# Autodesk Inventor assembly: PCB enclosure_v2
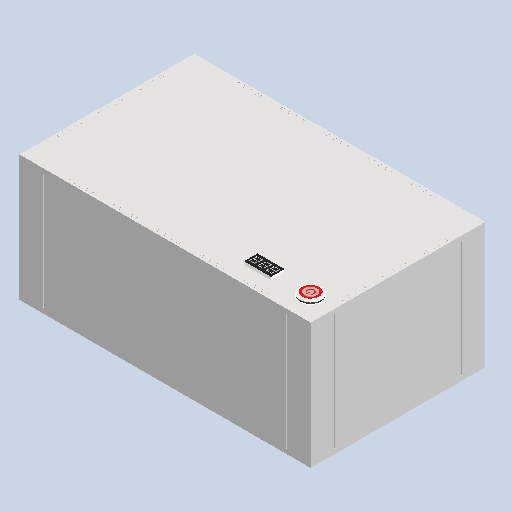
[picture p0: Inventor's stored thumbnail of the model, 512x512]
Saved by Autodesk Inventor 2026 (Build 300175050, 175E)
## iProperties
Created: 2025-10-28
Part Number: PCB enclosure_v2
Document SubType Name: Assembly
Designer: Kartik
Mass: 882.1 g
Surface Area: 6140.05 cm^2
Volume: 881.115 cm^3
Density: 1.00112 g/cm^3
Author: Kartik
## Documents named in this file (18)
- D:\Kartik\Projects\AMR\CAD\2 Sub-assembly\PCB enclosure_v2.iam
- D:\Kartik\Projects\AMR\CAD\4 Boughtouts\MDD20A CAD\MDD20A\MDD20A\MDD20A.ipt
- D:\Kartik\Projects\AMR\CAD\4 Boughtouts\NUCLEO-F401RE--3DModel-STEP-56544\NUCLEO-F401RE--3DModel-STEP-56544\NUCLEO-F401RE--3DModel-STEP-56544.ipt
- D:\Kartik\Projects\AMR\CAD\4 Boughtouts\nvidia-jetson-nano-4gb\Jetson nano 4GB\Jetson nano 4GB\Jetson nano 4GB.ipt
- D:\Kartik\Projects\AMR\CAD\4 Boughtouts\arduino-uno-screw-shield-1\Arduino Uno Screw Shield\Arduino Uno Screw Shield\Arduino Uno Screw Shield.ipt
- D:\Kartik\Projects\AMR\CAD\4 Boughtouts\xh-m401-buck-converter\XH-M401 Buck converter (XL4016E1)\XH-M401 Buck converter (XL4016E1)\XH-M401 Buck converter (XL4016E1).ipt
- D:\Kartik\Projects\AMR\CAD\4 Boughtouts\LM2596 DC-DC StepDown Converter v1\LM2596 DC-DC StepDown Converter v1\LM2596 DC-DC StepDown Converter v1.ipt
- D:\Kartik\Projects\AMR\CAD\4 Boughtouts\push-button-16-mm-led-1\LED_Button16mm\LED_Button_16mm\LED_Button_16mm\LED_Button_16mm.ipt
- D:\Kartik\Projects\AMR\CAD\4 Boughtouts\electrical-part-fuse-holder\Fuse Holder - CONQUER CQ-201N_.iam
- D:\Kartik\Projects\AMR\CAD\3 Parts\Enclosure_1.ipt
- D:\Kartik\Projects\AMR\CAD\4 Boughtouts\volt-meter-led-display-1\LED Display v3\LED Display v3\LED Display v3.ipt
- D:\Kartik\Projects\AMR\CAD\3 Parts\Enclosure_2.ipt
- D:\Kartik\Projects\AMR\CAD\3 Parts\Enclosure_4.ipt
- D:\Kartik\Projects\AMR\CAD\3 Parts\Enclosure_3.ipt
- D:\Kartik\Projects\AMR\CAD\3 Parts\Enclosure_5.ipt
- D:\Kartik\Projects\AMR\CAD\3 Parts\Enclosure_6.ipt
- D:\Kartik\Projects\AMR\CAD\3 Parts\Enclosure_7.ipt
- D:\Kartik\Projects\AMR\CAD\4 Boughtouts\volt-meter-led-display-1\LED Display v3\Amass XT60E1-M v4.ipt
## Components (17 placed, 17 different names)
1. MDD20A:1 — Mate:1, Flush:11, Mate:30, Angle:3, Flush:16
2. NUCLEO-F401RE--3DModel-STEP-56544:1 — Mate:1, Flush:9, Mate:6, Mate:25, Mate:26, Mate:27
3. Jetson nano 4GB:1 — Flush:9, Angle:1, Mate:31
4. Arduino Uno Screw Shield:1 — Mate:25, Mate:26, Mate:27
5. XH-M401 Buck converter (XL4016E1):1 — Flush:11, Flush:13, Angle:2
6. LM2596 DC-DC StepDown Converter v1:1 — Flush:13
7. LED_Button_16mm:1 — Mate:29, Flush:17, Mate:41, Flush:24
8. Fuse Holder - CONQUER CQ-201N_:2 [sub-assembly] — Angle:2, Mate:29
9. Enclosure_1:1 — Mate:30, Angle:3, Flush:16, Mate:31, Mate:32, Flush:18, Mate:33, Mate:34, Flush:19, Mate:35, Mate:36, Mate:37, Flush:20, Mate:38, Mate:39, Flush:21, Mate:40, Flush:23, Mate:46
10. LED Display v3:1 — Flush:17, Mate:42, Mate:43
11. Enclosure_2:1 — Mate:32, Flush:18, Mate:33, Flush:22, Mate:47
12. Enclosure_3:1 — Mate:34, Flush:19, Mate:35, Mate:44
13. Enclosure_4:1 — Mate:36, Mate:37, Flush:20
14. Enclosure_5:1 — Mate:38, Mate:39, Flush:21, Mate:45
15. Enclosure_6:1 — Mate:40, Flush:22, Flush:23, Mate:41, Flush:24, Mate:42, Mate:43
16. Enclosure_7:1 — Mate:44, Mate:45, Mate:46
17. Amass XT60E1-M v4:1 — Mate:47
## Relationships (40: Mate 24, Flush 13, Angle 3)
- Mate:1 (50 mm): MDD20A:1 ↔ NUCLEO-F401RE--3DModel-STEP-56544:1
- Flush:9: NUCLEO-F401RE--3DModel-STEP-56544:1 ↔ Jetson nano 4GB:1
- Angle:1 (0 deg): Jetson nano 4GB:1
- Mate:6: NUCLEO-F401RE--3DModel-STEP-56544:1
- Mate:25: NUCLEO-F401RE--3DModel-STEP-56544:1 ↔ Arduino Uno Screw Shield:1
- Mate:26: NUCLEO-F401RE--3DModel-STEP-56544:1 ↔ Arduino Uno Screw Shield:1
- Mate:27: NUCLEO-F401RE--3DModel-STEP-56544:1 ↔ Arduino Uno Screw Shield:1
- [Flush]: XH-M401 Buck converter (XL4016E1):1 ↔ LM2596 DC-DC StepDown Converter v1:1
- Flush:11: MDD20A:1 ↔ XH-M401 Buck converter (XL4016E1):1
- Flush:13: XH-M401 Buck converter (XL4016E1):1 ↔ LM2596 DC-DC StepDown Converter v1:1
- Angle:2 (90 deg): XH-M401 Buck converter (XL4016E1):1 ↔ Fuse Holder - CONQUER CQ-201N_:2
- Mate:29: LED_Button_16mm:1 ↔ Fuse Holder - CONQUER CQ-201N_:2
- Mate:30 (7 mm): MDD20A:1 ↔ Enclosure_1:1
- Angle:3 (0 deg): MDD20A:1 ↔ Enclosure_1:1
- Flush:16 (10 mm): MDD20A:1 ↔ Enclosure_1:1
- Mate:31: Jetson nano 4GB:1 ↔ Enclosure_1:1
- Flush:17: LED_Button_16mm:1 ↔ LED Display v3:1
- Mate:32: Enclosure_1:1 ↔ Enclosure_2:1
- Flush:18: Enclosure_1:1 ↔ Enclosure_2:1
- Mate:33 (1 mm): Enclosure_1:1 ↔ Enclosure_2:1
- Mate:34: Enclosure_1:1 ↔ Enclosure_3:1
- Flush:19: Enclosure_1:1 ↔ Enclosure_3:1
- Mate:35 (1 mm): Enclosure_1:1 ↔ Enclosure_3:1
- Mate:36: Enclosure_1:1 ↔ Enclosure_4:1
- Mate:37 (1 mm): Enclosure_1:1 ↔ Enclosure_4:1
- Flush:20: Enclosure_1:1 ↔ Enclosure_4:1
- Mate:38: Enclosure_1:1 ↔ Enclosure_5:1
- Mate:39 (1 mm): Enclosure_1:1 ↔ Enclosure_5:1
- Flush:21: Enclosure_1:1 ↔ Enclosure_5:1
- Mate:40: Enclosure_1:1 ↔ Enclosure_6:1
- Flush:22: Enclosure_2:1 ↔ Enclosure_6:1
- Flush:23: Enclosure_1:1 ↔ Enclosure_6:1
- Mate:41: LED_Button_16mm:1 ↔ Enclosure_6:1
- Flush:24: LED_Button_16mm:1 ↔ Enclosure_6:1
- Mate:42: LED Display v3:1 ↔ Enclosure_6:1
- Mate:43: LED Display v3:1 ↔ Enclosure_6:1
- Mate:44 (0.1 mm): Enclosure_3:1 ↔ Enclosure_7:1
- Mate:45 (0.1 mm): Enclosure_5:1 ↔ Enclosure_7:1
- Mate:46: Enclosure_1:1 ↔ Enclosure_7:1
- Mate:47: Enclosure_2:1 ↔ Amass XT60E1-M v4:1
